# Autodesk Inventor assembly: Übertragung des Zahnriemens
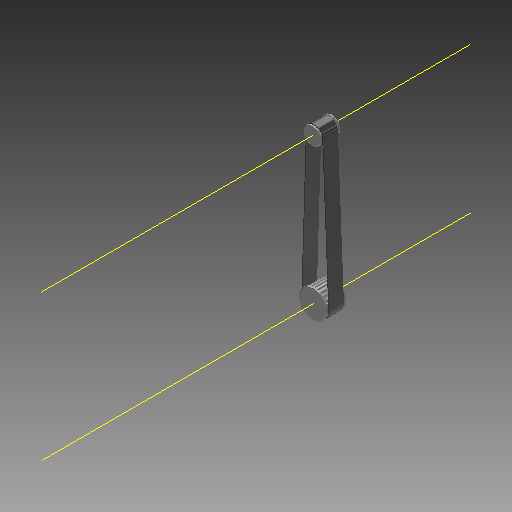
[picture p0: Inventor's stored thumbnail of the model, 512x512]
Saved by Autodesk Inventor 2019 (Build 230136000, 136)
## iProperties
ClientObjectVersion: 1
Created: 2021-04-25
Part Number: Übertragung des Zahnriemens
Document SubType Name: Assembly
Designer: Michael Sumper
Author: Michael Sumper
## Documents named in this file (4)
- C:\Users\Michael Sumper\OneDrive\Documents\Inventor\Portalfräse Devil'sCNC\Tower\Konstruktions-Assistent\Übertragung des Zahnriemens1.iam
- C:\Users\Michael Sumper\OneDrive\Documents\Inventor\Portalfräse Devil'sCNC\Tower\Konstruktions-Assistent\Zahnriemen1.ipt
- C:\Users\Michael Sumper\OneDrive\Documents\Inventor\Portalfräse Devil'sCNC\Tower\Konstruktions-Assistent\Synchrone Riemenscheibe11.ipt
- C:\Users\Michael Sumper\OneDrive\Documents\Inventor\Portalfräse Devil'sCNC\Tower\Konstruktions-Assistent\Synchrone Riemenscheibe21.ipt
## Components (3 placed, 3 different names)
1. Zahnriemen:1 — Fluchtend:1, Passend:1, Passend:2, Fluchtend:2, Passend:3, Passend:4
2. Synchrone Riemenscheibe1:1 — Fluchtend:1, Passend:1, Passend:2, Drehung:1
3. Synchrone Riemenscheibe2:1 — Fluchtend:2, Passend:3, Drehung:1, Passend:4
## Relationships (7: Mate 4, Flush 2, RelateRotation 1)
- Fluchtend:1 [Flush]: Zahnriemen:1 ↔ Synchrone Riemenscheibe1:1
- Passend:1 [Mate]: Zahnriemen:1 ↔ Synchrone Riemenscheibe1:1
- Passend:2 [Mate]: Zahnriemen:1 ↔ Synchrone Riemenscheibe1:1
- Fluchtend:2 [Flush]: Zahnriemen:1 ↔ Synchrone Riemenscheibe2:1
- Passend:3 [Mate]: Zahnriemen:1 ↔ Synchrone Riemenscheibe2:1
- Drehung:1 [RelateRotation] (1.6429 ul): Synchrone Riemenscheibe1:1 ↔ Synchrone Riemenscheibe2:1
- Passend:4 [Mate]: Zahnriemen:1 ↔ Synchrone Riemenscheibe2:1
